# Autodesk Inventor assembly: linac_mover_upper_ax_holder-asm
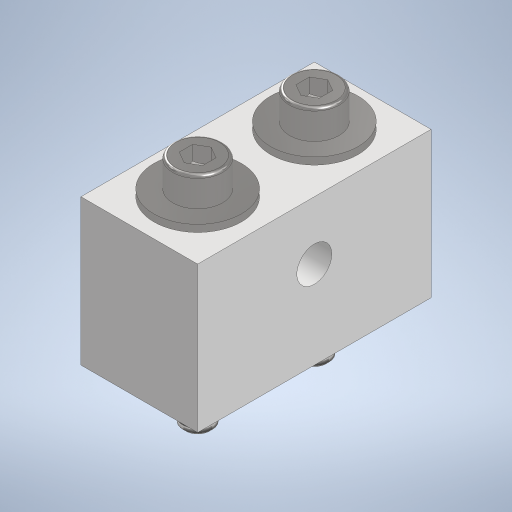
[picture p0: Inventor's stored thumbnail of the model, 512x512]
Saved by Autodesk Inventor 2024 (Build 280153000, 153)
## iProperties
Created: 2025-12-26
Part Number: linac_mover_upper_ax_holder-asm
Document SubType Name: Assembly
Designer: schar
Author: schar
## Documents named in this file (6)
- C:\Users\schar\Desktop\projectBlueprint\AMSTS\hardware\linac_mover_upper_ax_holder-asm.iam
- C:\Users\schar\Desktop\projectBlueprint\AMSTS\hardware\linac_mover_upper_ax_holder.ipt
- C:\Users\schar\Documents\Inventor\Content Center Files\R2024\en-US\DIN 9021\DIN 9021 - 5,3.ipt
- C:\Users\schar\Documents\Inventor\Content Center Files\R2024\en-US\ISO 4762(1)\DIN EN ISO 4762 - M5 x 35.ipt
- C:\Users\schar\Desktop\projectBlueprint\AMSTS\hardware\tnut_m5_2020.ipt
- C:\Users\schar\Desktop\projectBlueprint\AMSTS\hardware\625.ipt
## Components (8 placed, 5 different names)
1. linac_mover_upper_ax_holder:1 — Mate:1, Mate:2, Mate:3, Mate:4, Mate:7, Mate:8, Rigid:1, Rigid:2, Mate:9, Mate:10
2. DIN 9021 5,3:1 — Mate:1, Mate:4, Mate:5
3. DIN 9021 5,3:2 — Mate:2, Mate:3, Mate:6
4. DIN EN ISO 4762 M5 x 35:1 — Mate:6, Mate:8
5. DIN EN ISO 4762 M5 x 35:2 — Mate:5, Mate:7
6. tnut_m5_2020:1 — Rigid:2
7. tnut_m5_2020:2 — Rigid:1
8. 625:1 — Mate:9, Mate:10
## Relationships (12: Mate 10, WeldJoint 2)
- Mate:1: linac_mover_upper_ax_holder:1 ↔ DIN 9021 5,3:1
- Mate:2: linac_mover_upper_ax_holder:1 ↔ DIN 9021 5,3:2
- Mate:3: linac_mover_upper_ax_holder:1 ↔ DIN 9021 5,3:2
- Mate:4: linac_mover_upper_ax_holder:1 ↔ DIN 9021 5,3:1
- Mate:5: DIN 9021 5,3:1 ↔ DIN EN ISO 4762 M5 x 35:2
- Mate:6: DIN 9021 5,3:2 ↔ DIN EN ISO 4762 M5 x 35:1
- Mate:7: linac_mover_upper_ax_holder:1 ↔ DIN EN ISO 4762 M5 x 35:2
- Mate:8: linac_mover_upper_ax_holder:1 ↔ DIN EN ISO 4762 M5 x 35:1
- Rigid:1 [WeldJoint] (-0.159 mm): linac_mover_upper_ax_holder:1 ↔ tnut_m5_2020:2
- Rigid:2 [WeldJoint] (-0.159 mm): linac_mover_upper_ax_holder:1 ↔ tnut_m5_2020:1
- Mate:9: linac_mover_upper_ax_holder:1 ↔ 625:1
- Mate:10: linac_mover_upper_ax_holder:1 ↔ 625:1
